# Autodesk Inventor assembly: deltabot
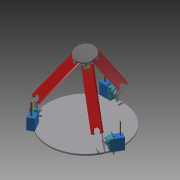
[picture p0: Inventor's stored thumbnail of the model, 180x180]
Saved by Autodesk Inventor 2015 SP2 (Build 190223200, 223)
## iProperties
Created: 2015-05-24
Part Number: deltabot
Document SubType Name: Assembly
Designer: caleb
Author: caleb
## Documents named in this file (7)
- C:\cygwin64\home\caleb\3d\designs\deep-focus-scanning-adapter\deltabot.iam
- C:\cygwin64\home\caleb\3d\designs\deep-focus-scanning-adapter\servo micro asm.iam
- C:\cygwin64\home\caleb\3d\designs\deep-focus-scanning-adapter\deltabot-table.ipt
- C:\cygwin64\home\caleb\3d\designs\deep-focus-scanning-adapter\ball bearing .5in.ipt
- C:\cygwin64\home\caleb\3d\designs\deep-focus-scanning-adapter\deltabot arm.ipt
- C:\cygwin64\home\caleb\3d\designs\deep-focus-scanning-adapter\deltabot base.ipt
- C:\cygwin64\home\caleb\3d\designs\deep-focus-scanning-adapter\servo micro asm2.iam
## Components (11 placed, 6 different names)
1. deltabot-table:1 — Mate:1
2. deltabot arm:1 — Mate:7, Mate:9
3. servo micro asm:1 [sub-assembly] — Mate:9, Mate:10, Mate:11, Flush:6
4. deltabot arm:2 — Mate:14, Mate:15
5. deltabot arm:3 — Mate:18, Mate:19
6. deltabot base:1 — Flush:3, Flush:4, Flush:5, Mate:10, Mate:11, Flush:6, Mate:12, Flush:7, Mate:13, Mate:16, Mate:17, Flush:8
7. servo micro asm2:1 [sub-assembly] — Mate:12, Flush:7, Mate:13, Mate:14
8. servo micro asm2:2 [sub-assembly] — Mate:16, Mate:17, Flush:8, Mate:19
9. ball bearing .5in:1 — Mate:1, Mate:7
10. ball bearing .5in:2 — Mate:18
11. ball bearing .5in:3 — Mate:15
## Component patterns: (3 elements, first: ball bearing .5in:1)
## Relationships (20: Mate 13, Flush 7)
- Mate:1: deltabot-table:1 ↔ ball bearing .5in:1
- Flush:1
- Mate:7: deltabot arm:1 ↔ ball bearing .5in:1
- Flush:3: deltabot base:1
- Flush:4: deltabot base:1
- Flush:5: deltabot base:1
- Mate:9: deltabot arm:1 ↔ servo micro asm:1
- Mate:10: servo micro asm:1 ↔ deltabot base:1
- Mate:11: servo micro asm:1 ↔ deltabot base:1
- Flush:6: servo micro asm:1 ↔ deltabot base:1
- Mate:12: deltabot base:1 ↔ servo micro asm2:1
- Flush:7: deltabot base:1 ↔ servo micro asm2:1
- Mate:13: deltabot base:1 ↔ servo micro asm2:1
- Mate:14: deltabot arm:2 ↔ servo micro asm2:1
- Mate:15: deltabot arm:2 ↔ ball bearing .5in:3
- Mate:16: deltabot base:1 ↔ servo micro asm2:2
- Mate:17: deltabot base:1 ↔ servo micro asm2:2
- Flush:8: deltabot base:1 ↔ servo micro asm2:2
- Mate:18: deltabot arm:3 ↔ ball bearing .5in:2
- Mate:19: deltabot arm:3 ↔ servo micro asm2:2
